# Autodesk Inventor assembly: Cover+Magnets
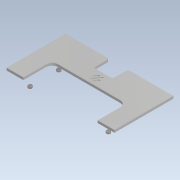
[picture p0: Inventor's stored thumbnail of the model, 180x180]
Saved by Autodesk Inventor 2022.1 (Build 261234020, 234B)
## iProperties
Created: 2022-07-24
Part Number: Cover+Magnets
Document SubType Name: Assembly
Designer: Rama
Author: Rama
## Documents named in this file (3)
- C:\Users\Rama\Desktop\GitHub\Voron-2-Mods\Mandalaroseworks\BedPan\CAD\SRC\Manual_Helpers\Cover+Magnets.iam
- C:\Users\Rama\Desktop\GitHub\Voron-2-Mods\Mandalaroseworks\BedPan\CAD\SRC\Cover\Cover.ipt
- C:\Users\Rama\Desktop\Work Priv\Klicky\6x3 Magnet.ipt
## Components (5 placed, 2 different names)
1. Cover:1 — Passend:1, Passend:2, Passend:3, Passend:4
2. 6x3 Magnet:1 — Passend:2
3. 6x3 Magnet:2 — Passend:3
4. 6x3 Magnet:3 — Passend:4
5. 6x3 Magnet:4 — Passend:1
## Relationships (7: Mate 4, Flush 3)
- [Flush]: 6x3 Magnet:2 ↔ 6x3 Magnet:3
- [Flush]: 6x3 Magnet:1 ↔ 6x3 Magnet:4
- [Flush]: 6x3 Magnet:3 ↔ 6x3 Magnet:4
- Passend:1 [Mate]: Cover:1 ↔ 6x3 Magnet:4
- Passend:2 [Mate]: Cover:1 ↔ 6x3 Magnet:1
- Passend:3 [Mate]: Cover:1 ↔ 6x3 Magnet:2
- Passend:4 [Mate]: Cover:1 ↔ 6x3 Magnet:3
